# Autodesk Inventor assembly: SPE42 Base Paciente
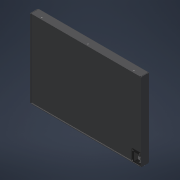
[picture p0: Inventor's stored thumbnail of the model, 180x180]
Saved by Autodesk Inventor 2021.2 (Build 252289000, 289)
## iProperties
Created: 2026-08-25
Part Number: SPE42 Base Paciente
Document SubType Name: Assembly
Designer: nelso
Mass: 16127.2 g
Surface Area: 31818.7 cm^2
Volume: 3944.79 cm^3
Density: 4.08822 g/cm^3
Author: nelso
## Documents named in this file (13)
- C:\Users\nelso\Documents\Escritorio\Soporte-Paciente-Espinografia\Workspace\SPE42 Base Paciente.iam
- C:\Users\nelso\Documents\Escritorio\Soporte-Paciente-Espinografia\Workspace\SP26V1 Base Chapa.ipt
- C:\Users\nelso\Documents\Escritorio\Soporte-Paciente-Espinografia\Workspace\SP32V1 Refuerzo.ipt
- C:\Users\nelso\Documents\Escritorio\Soporte-Paciente-Espinografia\Workspace\SP41V1 Cubre Base.ipt
- C:\Users\nelso\Documents\Escritorio\Soporte-Paciente-Espinografia\Workspace\RFPLUS4PO300 Tuerca rem M4 cab red.ipt
- C:\Users\nelso\Documents\Escritorio\Soporte-Paciente-Espinografia\Workspace\DIN7991M4X0.8L12C.ipt
- C:\Users\nelso\Documents\Escritorio\Soporte-Paciente-Espinografia\Workspace\SP41V1 Goma Base.ipt
- C:\Users\nelso\Documents\Escritorio\Soporte-Paciente-Espinografia\Workspace\SP40V1 Refuerzo pasador.ipt
- C:\Users\nelso\Documents\Escritorio\Soporte-Paciente-Espinografia\Workspace\SKU1009783 -PasadorSCMetalurgica58mm.iam
- C:\Users\nelso\Documents\Escritorio\Soporte-Paciente-Espinografia\Workspace\SP49V1 Protector Pasador.ipt
- C:\Users\nelso\Documents\Escritorio\Soporte-Paciente-Espinografia\Workspace\ISO7380M3X0.5L8I.ipt
- C:\Users\nelso\Documents\Escritorio\Soporte-Paciente-Espinografia\Workspace\DIN137-B3.ipt
- C:\Users\nelso\Documents\Escritorio\Soporte-Paciente-Espinografia\Workspace\DIN555-5M3X0.5I.ipt
## Components (29 placed, 12 different names)
1. SP26V1 Base Chapa:1 — Flush:14, Flush:15, Flush:16
2. SP32V1 Refuerzo:1
3. SP40V1 Refuerzo pasador:1 — Mate:31, Flush:13, Mate:32, Mate:33
4. SP32V1 Refuerzo:3
5. SP41V1 Cubre Base:1 — Mate:34, Mate:35, Mate:36, Mate:37, Mate:38, Mate:48, Mate:49, Mate:50
6. RFPLUS4PO300 Tuerca rem M4 cab red:1 — Mate:34
7. RFPLUS4PO300 Tuerca rem M4 cab red:2
8. RFPLUS4PO300 Tuerca rem M4 cab red:3
9. RFPLUS4PO300 Tuerca rem M4 cab red:4
10. RFPLUS4PO300 Tuerca rem M4 cab red:5
11. RFPLUS4PO300 Tuerca rem M4 cab red:6 — Mate:35
12. DIN7991M4X0.8L12C:1
13. DIN7991M4X0.8L12C:2
14. DIN7991M4X0.8L12C:3
15. DIN7991M4X0.8L12C:4
16. DIN7991M4X0.8L12C:5
17. DIN7991M4X0.8L12C:6
18. SP41V1 Goma Base:1
19. SKU1009783 -PasadorSCMetalurgica58mm:1 [sub-assembly] — Mate:31, Flush:13, Mate:32, Mate:33
20. SP49V1 Protector Pasador:1 — Mate:36, Mate:37, Mate:38, Mate:39, Mate:40, Mate:41, Mate:42, Mate:43, Mate:44
21. ISO7380M3X0.5L8I:1 — Mate:40, Mate:44, Mate:46, Mate:56
22. ISO7380M3X0.5L8I:2 — Mate:39, Mate:42, Mate:47, Mate:52
23. ISO7380M3X0.5L8I:3 — Mate:41, Mate:43, Mate:45, Mate:54
24. DIN137-B3:1 — Mate:45, Mate:49, Mate:53
25. DIN137-B3:2 — Mate:46, Mate:50, Mate:55
26. DIN137-B3:3 — Mate:47, Mate:48, Mate:51
27. DIN555-5M3X0.5I:1 — Mate:53, Mate:54
28. DIN555-5M3X0.5I:2 — Mate:55, Mate:56
29. DIN555-5M3X0.5I:3 — Mate:51, Mate:52
## Relationships (68: Mate 53, Flush 15)
- [Mate]: SP26V1 Base Chapa:1 ↔ SP40V1 Refuerzo pasador:1
- [Mate]: SP26V1 Base Chapa:1 ↔ SP32V1 Refuerzo:3
- [Mate]: SP26V1 Base Chapa:1 ↔ SP32V1 Refuerzo:1
- [Mate]: SP26V1 Base Chapa:1 ↔ SP32V1 Refuerzo:3
- [Mate]: SP26V1 Base Chapa:1 ↔ SP40V1 Refuerzo pasador:1
- [Mate]: SP26V1 Base Chapa:1 ↔ SP32V1 Refuerzo:1
- [Flush]: SP26V1 Base Chapa:1 ↔ SP40V1 Refuerzo pasador:1
- [Flush]: SP26V1 Base Chapa:1 ↔ SP32V1 Refuerzo:1
- [Flush]: SP26V1 Base Chapa:1 ↔ SP32V1 Refuerzo:3
- [Flush]: SP26V1 Base Chapa:1 ↔ SP41V1 Cubre Base:1
- [Flush]: SP26V1 Base Chapa:1 ↔ SP41V1 Cubre Base:1
- [Mate]: SP26V1 Base Chapa:1 ↔ RFPLUS4PO300 Tuerca rem M4 cab red:6
- [Mate]: SP26V1 Base Chapa:1 ↔ RFPLUS4PO300 Tuerca rem M4 cab red:5
- [Mate]: SP26V1 Base Chapa:1 ↔ RFPLUS4PO300 Tuerca rem M4 cab red:4
- [Mate]: SP26V1 Base Chapa:1 ↔ RFPLUS4PO300 Tuerca rem M4 cab red:1
- [Mate]: SP26V1 Base Chapa:1 ↔ RFPLUS4PO300 Tuerca rem M4 cab red:2
- [Mate]: SP26V1 Base Chapa:1 ↔ RFPLUS4PO300 Tuerca rem M4 cab red:3
- [Mate]: SP26V1 Base Chapa:1 ↔ RFPLUS4PO300 Tuerca rem M4 cab red:1
- [Mate]: SP26V1 Base Chapa:1 ↔ RFPLUS4PO300 Tuerca rem M4 cab red:2
- [Mate]: SP26V1 Base Chapa:1 ↔ RFPLUS4PO300 Tuerca rem M4 cab red:3
- [Mate]: SP26V1 Base Chapa:1 ↔ RFPLUS4PO300 Tuerca rem M4 cab red:4
- [Mate]: SP26V1 Base Chapa:1 ↔ RFPLUS4PO300 Tuerca rem M4 cab red:5
- [Mate]: SP26V1 Base Chapa:1 ↔ RFPLUS4PO300 Tuerca rem M4 cab red:6
- [Mate]: SP26V1 Base Chapa:1 ↔ DIN7991M4X0.8L12C:1
- [Mate]: SP26V1 Base Chapa:1 ↔ DIN7991M4X0.8L12C:2
- [Mate]: SP26V1 Base Chapa:1 ↔ DIN7991M4X0.8L12C:3
- [Mate]: SP26V1 Base Chapa:1 ↔ DIN7991M4X0.8L12C:4
- [Mate]: SP26V1 Base Chapa:1 ↔ DIN7991M4X0.8L12C:5
- [Mate]: SP26V1 Base Chapa:1 ↔ DIN7991M4X0.8L12C:6
- [Flush]: SP26V1 Base Chapa:1 ↔ DIN7991M4X0.8L12C:3
- [Flush]: SP26V1 Base Chapa:1 ↔ DIN7991M4X0.8L12C:2
- [Flush]: SP26V1 Base Chapa:1 ↔ DIN7991M4X0.8L12C:1
- [Flush]: SP26V1 Base Chapa:1 ↔ DIN7991M4X0.8L12C:6
- [Flush]: SP26V1 Base Chapa:1 ↔ DIN7991M4X0.8L12C:5
- [Flush]: SP26V1 Base Chapa:1 ↔ DIN7991M4X0.8L12C:4
- [Mate]: SP26V1 Base Chapa:1 ↔ SP41V1 Goma Base:1
- [Mate]: SP26V1 Base Chapa:1 ↔ SP41V1 Goma Base:1
- [Mate]: SP26V1 Base Chapa:1 ↔ SP41V1 Goma Base:1
- Mate:31: SP40V1 Refuerzo pasador:1 ↔ SKU1009783 -PasadorSCMetalurgica58mm:1
- Flush:13: SP40V1 Refuerzo pasador:1 ↔ SKU1009783 -PasadorSCMetalurgica58mm:1
- Mate:32: SP40V1 Refuerzo pasador:1 ↔ SKU1009783 -PasadorSCMetalurgica58mm:1
- Mate:33: SP40V1 Refuerzo pasador:1 ↔ SKU1009783 -PasadorSCMetalurgica58mm:1
- Mate:34: SP41V1 Cubre Base:1 ↔ RFPLUS4PO300 Tuerca rem M4 cab red:1
- Mate:35: SP41V1 Cubre Base:1 ↔ RFPLUS4PO300 Tuerca rem M4 cab red:6
- Flush:14: SP26V1 Base Chapa:1
- Flush:15: SP26V1 Base Chapa:1
- Flush:16: SP26V1 Base Chapa:1
- Mate:36: SP41V1 Cubre Base:1 ↔ SP49V1 Protector Pasador:1
- Mate:37: SP41V1 Cubre Base:1 ↔ SP49V1 Protector Pasador:1
- Mate:38: SP41V1 Cubre Base:1 ↔ SP49V1 Protector Pasador:1
- Mate:39: SP49V1 Protector Pasador:1 ↔ ISO7380M3X0.5L8I:2
- Mate:40: SP49V1 Protector Pasador:1 ↔ ISO7380M3X0.5L8I:1
- Mate:41: SP49V1 Protector Pasador:1 ↔ ISO7380M3X0.5L8I:3
- Mate:42: SP49V1 Protector Pasador:1 ↔ ISO7380M3X0.5L8I:2
- Mate:43: SP49V1 Protector Pasador:1 ↔ ISO7380M3X0.5L8I:3
- Mate:44: SP49V1 Protector Pasador:1 ↔ ISO7380M3X0.5L8I:1
- Mate:45: ISO7380M3X0.5L8I:3 ↔ DIN137-B3:1
- Mate:46: ISO7380M3X0.5L8I:1 ↔ DIN137-B3:2
- Mate:47: ISO7380M3X0.5L8I:2 ↔ DIN137-B3:3
- Mate:48: SP41V1 Cubre Base:1 ↔ DIN137-B3:3
- Mate:49: SP41V1 Cubre Base:1 ↔ DIN137-B3:1
- Mate:50: SP41V1 Cubre Base:1 ↔ DIN137-B3:2
- Mate:51: DIN137-B3:3 ↔ DIN555-5M3X0.5I:3
- Mate:52: ISO7380M3X0.5L8I:2 ↔ DIN555-5M3X0.5I:3
- Mate:53: DIN137-B3:1 ↔ DIN555-5M3X0.5I:1
- Mate:54: ISO7380M3X0.5L8I:3 ↔ DIN555-5M3X0.5I:1
- Mate:55: DIN137-B3:2 ↔ DIN555-5M3X0.5I:2
- Mate:56: ISO7380M3X0.5L8I:1 ↔ DIN555-5M3X0.5I:2
